# Autodesk Inventor assembly: HållareV.2
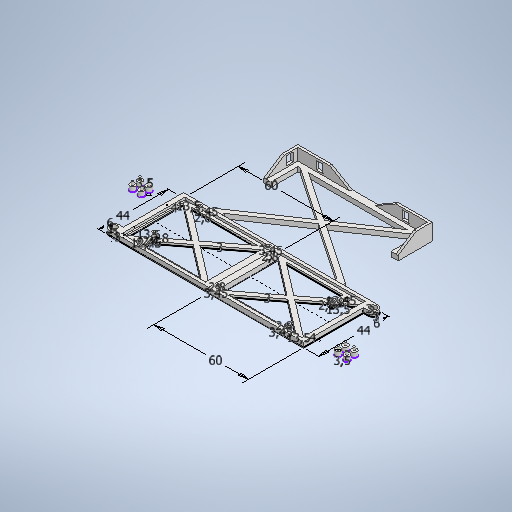
[picture p0: Inventor's stored thumbnail of the model, 512x512]
Saved by Autodesk Inventor 2025.2 (Build 292293000, 293)
## iProperties
Created: 2025-01-22
Part Number: HållareV.2
Document SubType Name: Assembly
Designer: 24oscnor
Author: 24oscnor
## Documents named in this file (3)
- C:\Users\24oscnor\programering\projects\skola\Wexteras\wextras\CAD\HållareV.2.iam
- C:\Users\24oscnor\programering\projects\skola\Wexteras\wextras\CAD\HållareV.2.ipt
- C:\Users\24oscnor\programering\projects\skola\Wexteras\wextras\CAD\Part6.ipt
## Components (3 placed, 2 different names)
1. HållareV.2:1 — Flush:1
2. HållareV.2:2 — Mate:2, Mate:12
3. Part6:1 — Flush:1, Mate:2, Mate:12
## Relationships (3: Mate 2, Flush 1)
- Flush:1: HållareV.2:1 ↔ Part6:1
- Mate:2 (19 mm): HållareV.2:2 ↔ Part6:1
- Mate:12: HållareV.2:2 ↔ Part6:1
